# Autodesk Inventor assembly: 8inWheel
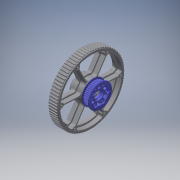
[picture p0: Inventor's stored thumbnail of the model, 180x180]
Saved by Autodesk Inventor 2016 (Build 200138000, 138)
## iProperties
Created: 2016-01-27
Part Number: 8inWheel
Document SubType Name: Assembly
Designer: 17swamipr
Author: 17swamipr
## Documents named in this file (3)
- C:\Users\17swamipr\Desktop\Robot Assembly\Special Assemblies\8inWheel.iam
- C:\Users\17swamipr\Desktop\Robot Assembly\Drive Train\8PlactionRough-500bearing.iam
- C:\Users\17swamipr\Desktop\Robot Assembly\Drive Train\am-2234_42toothHTDpulleyHalfRev2.ipt
## Components (3 placed, 2 different names)
1. 8PlactionRough-500bearing:1 [sub-assembly] — Mate:1, Mate:2, Mate:3
2. am-2234_42toothHTDpulleyHalfRev2:1 — Mate:1, Mate:2, Mate:3, Insert:1, Insert:2
3. am-2234_42toothHTDpulleyHalfRev2:2 — Insert:1, Insert:2
## Relationships (5: Mate 3, Insert 2)
- Mate:1: 8PlactionRough-500bearing:1 ↔ am-2234_42toothHTDpulleyHalfRev2:1
- Mate:2: 8PlactionRough-500bearing:1 ↔ am-2234_42toothHTDpulleyHalfRev2:1
- Mate:3: 8PlactionRough-500bearing:1 ↔ am-2234_42toothHTDpulleyHalfRev2:1
- Insert:1: am-2234_42toothHTDpulleyHalfRev2:1 ↔ am-2234_42toothHTDpulleyHalfRev2:2
- Insert:2: am-2234_42toothHTDpulleyHalfRev2:1 ↔ am-2234_42toothHTDpulleyHalfRev2:2
